# Autodesk Inventor assembly: ZŁĄCZA + BLACHA
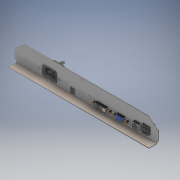
[picture p0: Inventor's stored thumbnail of the model, 180x180]
Saved by Autodesk Inventor 2017 SP1 (Build 210196100, 196)
## iProperties
Created: 2021-02-21
Part Number: ZŁĄCZA + BLACHA
Document SubType Name: Assembly
Designer: Napoleon
Author: Napoleon
## Documents named in this file (10)
- D:\PRYWATNE\PROJEKTY\POKÓJ\URZĄDZENIA PERYFERYJNE\DELL 1909Wf\BLACHA+ZŁĄCZA.iam
- D:\PRYWATNE\PROJEKTY\POKÓJ\URZĄDZENIA PERYFERYJNE\DELL 1909Wf\BLACHA OBUDOWY TYLNEJ MONITORA.ipt
- D:\PRYWATNE\PROJEKTY\POKÓJ\URZĄDZENIA PERYFERYJNE\DELL 1909Wf\ZŁĄCZA\IEC C14.ipt
- D:\PRYWATNE\PROJEKTY\POKÓJ\URZĄDZENIA PERYFERYJNE\DELL 1909Wf\ZŁĄCZA\AUDIO DC12.ipt
- D:\PRYWATNE\PROJEKTY\POKÓJ\URZĄDZENIA PERYFERYJNE\DELL 1909Wf\ZŁĄCZA\DVI.ipt
- D:\PRYWATNE\PROJEKTY\POKÓJ\URZĄDZENIA PERYFERYJNE\DELL 1909Wf\ZŁĄCZA\D-SUB.ipt
- C:\Users\Administrator\Documents\Inventor\Content Center Files\R2017\pl-PL\AS 1427(04)\AS 1427 - M3 x 5(5) I.ipt
- D:\PRYWATNE\PROJEKTY\POKÓJ\URZĄDZENIA PERYFERYJNE\DELL 1909Wf\ZŁĄCZA\USB B\USB Series B Receptacle.iam
- D:\PRYWATNE\PROJEKTY\POKÓJ\URZĄDZENIA PERYFERYJNE\DELL 1909Wf\ZŁĄCZA\USB A 2.0\femaleThruHoleUSB.ipt
- D:\PRYWATNE\PROJEKTY\POKÓJ\URZĄDZENIA PERYFERYJNE\DELL 1909Wf\ZŁĄCZA\ŚRUBA DO ZŁĄCZ.ipt
## Components (14 placed, 9 different names)
1. BLACHA OBUDOWY TYLNEJ MONITORA:1 — Zestawiający:3, Zestawiający:4, Zestawiający:5, Zestawiający:6, Zestawiający:7, Równoległy:1, Zestawiający:8, Zestawiający:9, Zestawiający:10, Zestawiający:20, Zestawiający:21, Równoległy:2, Zestawiający:24, Zestawiający:25, Zestawiający:26, Zestawiający:27, Zestawiający:28, Zestawiający:30, Walcowe:1, Walcowe:2, Walcowe:3, Walcowe:4
2. IEC C14:1 — Zestawiający:3, Zestawiający:4, Zestawiający:5
3. AUDIO DC12:1 — Zestawiający:6, Zestawiający:7, Równoległy:1
4. DVI:1 — Zestawiający:8, Zestawiający:9, Zestawiający:10
5. D-SUB:1 — Zestawiający:30
6. AS 1427 H - Metryczny M3 x 5:1
7. AS 1427 H - Metryczny M3 x 5:2
8. femaleThruHoleUSB:1 — Zestawiający:24, Zestawiający:25, Zestawiający:26, Zestawiający:29
9. USB Series B Receptacle:1 [sub-assembly] — Zestawiający:20, Zestawiający:21, Równoległy:2
10. femaleThruHoleUSB:2 — Zestawiający:27, Zestawiający:28, Zestawiający:29
11. ŚRUBA DO ZŁĄCZ:1 — Walcowe:4
12. ŚRUBA DO ZŁĄCZ:2 — Walcowe:3
13. ŚRUBA DO ZŁĄCZ:3 — Walcowe:2
14. ŚRUBA DO ZŁĄCZ:4 — Walcowe:1
## Relationships (23: Mate 17, CylindricalJoint 4, Flush 2)
- Zestawiający:3 [Mate]: BLACHA OBUDOWY TYLNEJ MONITORA:1 ↔ IEC C14:1
- Zestawiający:4 [Mate] (0.5 mm): BLACHA OBUDOWY TYLNEJ MONITORA:1 ↔ IEC C14:1
- Zestawiający:5 [Mate] (0.5 mm): BLACHA OBUDOWY TYLNEJ MONITORA:1 ↔ IEC C14:1
- Zestawiający:6 [Mate] (0.25 mm): BLACHA OBUDOWY TYLNEJ MONITORA:1 ↔ AUDIO DC12:1
- Zestawiający:7 [Mate] (0.25 mm): BLACHA OBUDOWY TYLNEJ MONITORA:1 ↔ AUDIO DC12:1
- Równoległy:1 [Flush] (-0.5 mm): BLACHA OBUDOWY TYLNEJ MONITORA:1 ↔ AUDIO DC12:1
- Zestawiający:8 [Mate] (0.25 mm): BLACHA OBUDOWY TYLNEJ MONITORA:1 ↔ DVI:1
- Zestawiający:9 [Mate] (0.25 mm): BLACHA OBUDOWY TYLNEJ MONITORA:1 ↔ DVI:1
- Zestawiający:10 [Mate]: BLACHA OBUDOWY TYLNEJ MONITORA:1 ↔ DVI:1
- Zestawiający:20 [Mate] (0.25 mm): BLACHA OBUDOWY TYLNEJ MONITORA:1 ↔ USB Series B Receptacle:1
- Zestawiający:21 [Mate] (0.25 mm): BLACHA OBUDOWY TYLNEJ MONITORA:1 ↔ USB Series B Receptacle:1
- Równoległy:2 [Flush] (-5 mm): BLACHA OBUDOWY TYLNEJ MONITORA:1 ↔ USB Series B Receptacle:1
- Zestawiający:24 [Mate] (3.5 mm): BLACHA OBUDOWY TYLNEJ MONITORA:1 ↔ femaleThruHoleUSB:1
- Zestawiający:25 [Mate]: BLACHA OBUDOWY TYLNEJ MONITORA:1 ↔ femaleThruHoleUSB:1
- Zestawiający:26 [Mate] (1.07 mm): BLACHA OBUDOWY TYLNEJ MONITORA:1 ↔ femaleThruHoleUSB:1
- Zestawiający:27 [Mate] (3.5 mm): BLACHA OBUDOWY TYLNEJ MONITORA:1 ↔ femaleThruHoleUSB:2
- Zestawiający:28 [Mate] (1.07 mm): BLACHA OBUDOWY TYLNEJ MONITORA:1 ↔ femaleThruHoleUSB:2
- Zestawiający:29 [Mate]: femaleThruHoleUSB:1 ↔ femaleThruHoleUSB:2
- Zestawiający:30 [Mate]: BLACHA OBUDOWY TYLNEJ MONITORA:1 ↔ D-SUB:1
- Walcowe:1 [CylindricalJoint]: BLACHA OBUDOWY TYLNEJ MONITORA:1 ↔ ŚRUBA DO ZŁĄCZ:4
- Walcowe:2 [CylindricalJoint]: BLACHA OBUDOWY TYLNEJ MONITORA:1 ↔ ŚRUBA DO ZŁĄCZ:3
- Walcowe:3 [CylindricalJoint]: BLACHA OBUDOWY TYLNEJ MONITORA:1 ↔ ŚRUBA DO ZŁĄCZ:2
- Walcowe:4 [CylindricalJoint]: BLACHA OBUDOWY TYLNEJ MONITORA:1 ↔ ŚRUBA DO ZŁĄCZ:1
